# Autodesk Inventor assembly: Piston Assembly
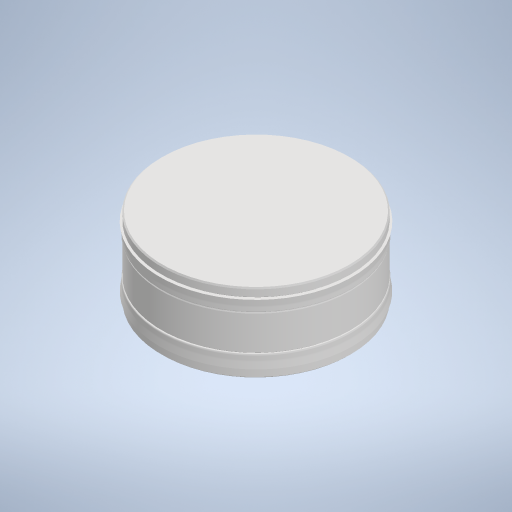
[picture p0: Inventor's stored thumbnail of the model, 512x512]
Saved by Autodesk Inventor 2024 (Build 280153000, 153)
## iProperties
Created: 2024-04-17
Part Number: Piston Assembly
Document SubType Name: Assembly
Designer: Tommy Rohmann
Author: Tommy Rohmann
## Documents named in this file (3)
- C:\Users\Tommy Rohmann\Documents\Repositories\Microgravity-Press-Washing-Machine\Sub-System Design and Documentation\Piston Assembly\Piston Assembly.iam
- C:\Users\Tommy Rohmann\Documents\Repositories\Microgravity-Press-Washing-Machine\Sub-System Design and Documentation\Piston Assembly\1 Piston Seal 4 OD O-Ring-Loaded U-Cup Seal.ipt
- C:\Users\Tommy Rohmann\Documents\Repositories\Microgravity-Press-Washing-Machine\Sub-System Design and Documentation\Piston Assembly\2 Piston.ipt
## Components (3 placed, 2 different names)
1. 1 Piston Seal 4 OD O-Ring-Loaded U-Cup Seal:1 — Mate:2, Mate:3
2. 1 Piston Seal 4 OD O-Ring-Loaded U-Cup Seal:2 — Mate:1, Mate:4
3. 2 Piston:1 — Mate:1, Mate:2, Mate:3, Mate:4
## Relationships (4: Mate 4)
- Mate:1: 1 Piston Seal 4 OD O-Ring-Loaded U-Cup Seal:2 ↔ 2 Piston:1
- Mate:2: 1 Piston Seal 4 OD O-Ring-Loaded U-Cup Seal:1 ↔ 2 Piston:1
- Mate:3: 1 Piston Seal 4 OD O-Ring-Loaded U-Cup Seal:1 ↔ 2 Piston:1
- Mate:4: 1 Piston Seal 4 OD O-Ring-Loaded U-Cup Seal:2 ↔ 2 Piston:1
